# Autodesk Inventor assembly: 2 Flex, HS
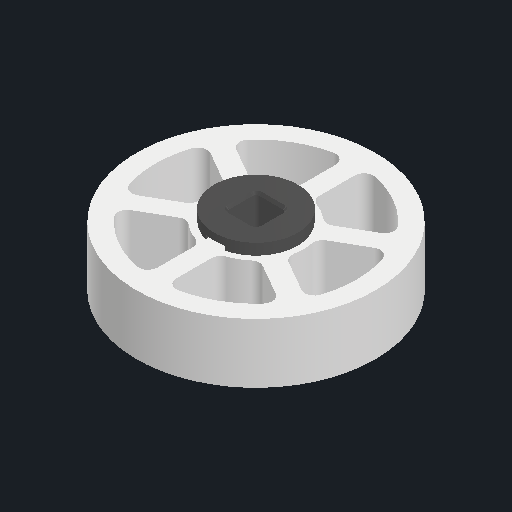
[picture p0: Inventor's stored thumbnail of the model, 512x512]
Saved by Autodesk Inventor 2024 (Build 280153000, 153)
## iProperties
Created: 2023-02-19
Part Number: 2 Flex, HS
Document SubType Name: Assembly
Designer: Windows Macbook
Author: Windows Macbook
## Documents named in this file (4)
- \\Mac\Home\Desktop\code\7899V-VRC-OVER-UNDER\Cad\VEX-CAD-Inventor-1.4.0\Motion\Wheels\Flex Wheels\2 Flex, HS.iam
- \\Mac\Home\Desktop\code\7899V-VRC-OVER-UNDER\Cad\VEX-CAD-Inventor-1.4.0\Motion\Wheels\Flex Wheels\2.000 Flex Wheel\2.000 30A .500.ipt
- C:\Users\Windows Macbook\Desktop\Inventor\Motion\Wheels\Flex Wheels\2.000 Flex Wheel.ipt
- \\Mac\Home\Desktop\code\7899V-VRC-OVER-UNDER\Cad\VEX-CAD-Inventor-1.4.0\Motion\Wheels\Flex Wheels\VersaHex Adapters .250.ipt
## Components (3 placed, 2 different names)
1. 2.000 30A .500:1 — Insert:1, Insert:2, Angle:1
2. VersaHex Adapters .250:1 — Insert:2, Angle:2
3. VersaHex Adapters .250:3 — Insert:1, Angle:1, Angle:2
## Relationships (4: Insert 2, Angle 2)
- Insert:1: 2.000 30A .500:1 ↔ VersaHex Adapters .250:3
- Insert:2: 2.000 30A .500:1 ↔ VersaHex Adapters .250:1
- Angle:1 (0 deg): 2.000 30A .500:1 ↔ VersaHex Adapters .250:3
- Angle:2 (0 deg): VersaHex Adapters .250:1 ↔ VersaHex Adapters .250:3
